# Autodesk Inventor assembly: BG003_huenin20_23
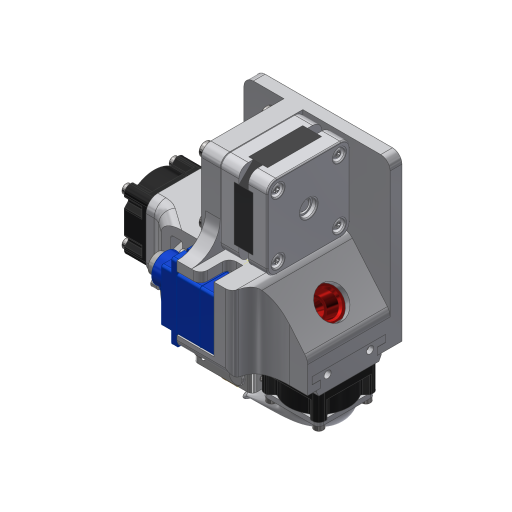
[picture p0: Inventor's stored thumbnail of the model, 512x512]
Saved by Autodesk Inventor 2023.3 (Build 273359000, 359)
## iProperties
Company: HTBLA Kaindorf
RuleStatus: InUse
Created: 2023-11-21
Part Number: BG003_huenin20_23
Project: Fiberprinter-Hotend
Material: Generisch
Description: Toolhead
Document SubType Name: Assembly
Designer: huenin20
Mass: 244.84 g
Surface Area: 631.325 cm^2
Volume: 123.223 cm^3
Density: 1.98697 g/cm^3
AfterDocNew0: iProperties-Editor_aufrufen
Author: nicob
Keywords: 2023
## Documents named in this file (17)
- H:\Dokumente\Projects\Kop\Fiberprinter_Hotend\BG003_huenin20_23_Fiberprinter-Hotend_Toolhead.iam
- H:\Dokumente\Projects\Kop\Fiberprinter_Hotend\BT010_huenin20_23_Fiberprinter-Hotend_hotendmount.ipt
- H:\Dokumente\Projects\Kop\Fiberprinter_Hotend\BT012_huenin20_23_Fiberprinter-Hotend_Faservorschubrad.ipt
- H:\Dokumente\Projects\Kop\Fiberprinter_Hotend\BT013_huenin20_23_Fiberprinter-Hotend_Faserführungsrad.ipt
- H:\Dokumente\Projects\Kop\Fiberprinter_Hotend\BT014_huenin20_23_Fiberprinter-Hotend_Faservorschubgleitlager.ipt
- H:\Dokumente\Projects\Kop\Fiberprinter_Hotend\BG001_huenin20_23_Fiberprinter-Hotend_Fiberprinter_Hotend.iam
- H:\Dokumente\Projects\Kop\Fiberprinter_Hotend\Step_downloads\Motoren\14HS08-0404S\14HS08-0404S.ipt
- H:\Dokumente\Projects\Kop\Fiberprinter_Hotend\Normteile\de-DE\ISO 2338(2)\ISO 2338 - 3 h8 x 8.ipt
- H:\Dokumente\Projects\Kop\Fiberprinter_Hotend\Step_downloads\25x25x10_fan\25x25x10_fan.ipt
- H:\Dokumente\Projects\Kop\Fiberprinter_Hotend\Step_downloads\Motoren\Servo\Servo.ipt
- H:\Dokumente\Projects\Kop\Fiberprinter_Hotend\Kurvenscheibe1.ipt
- H:\Dokumente\Projects\Kop\Fiberprinter_Hotend\Normteile\de-DE\DIN 912\DIN 912 - M3 x 0,5 x 12 x 10,75.ipt
- H:\Dokumente\Projects\Kop\Fiberprinter_Hotend\Normteile\de-DE\DIN 912\DIN 912 - M3 x 0,5 x 6 x 4,75.ipt
- H:\Dokumente\Projects\Kop\Fiberprinter_Hotend\Normteile\de-DE\ISO 4762(2)\ISO 4762 - M1,6 x 6ISO.ipt
- H:\Dokumente\Projects\Kop\Fiberprinter_Hotend\BT016_huenin20_24_Fiberprinter-Hotend_Bauteilkühllüfter_befestigung.ipt
- H:\Dokumente\Projects\Kop\Fiberprinter_Hotend\BT017_huenin20_24_Fiberprinter-Hotend_Bauteillüfterkanal.ipt
- H:\Dokumente\Projects\Kop\Fiberprinter_Hotend\Normteile\de-DE\DIN 912\DIN 912 - M2 x 0,4 x 16 x 15.ipt
## Components (30 placed, 16 different names)
1. BG001_huenin20_23_Fiberprinter-Hotend_Fiberprinter_Hotend:1 [sub-assembly] — Einfügen:61, Winkel:1, Passend:11, Winkel:2
2. DIN 912 - ersetzt durch DIN EN ISO 4762 M3 x 12:2 — Einfügen:63
3. DIN 912 - ersetzt durch DIN EN ISO 4762 M3 x 12:1 — Einfügen:62
4. DIN 912 - ersetzt durch DIN EN ISO 4762 M3 x 6:1 — Einfügen:58
5. BT010_huenin20_23_Fiberprinter-Hotend_hotendmount:1 — Einfügen:39, Einfügen:40, Einfügen:43, Einfügen:52, Einfügen:53, Einfügen:58, Einfügen:59, Einfügen:60, Einfügen:61, Winkel:1, Einfügen:62, Einfügen:63, Einfügen:64, Einfügen:65, Einfügen:66, Einfügen:67, Passend:7, Passend:8, Fluchtend:2
6. ISO 4762 M1,6 x 6:2 — Einfügen:73
7. ISO 4762 M1,6 x 6:1 — Einfügen:72
8. Servo:1 — Passend:4, Passend:5, Einfügen:59, Einfügen:60, Einfügen:72, Einfügen:73
9. Kurvenscheibe:1 — Passend:4, Passend:5
10. DIN 912 - ersetzt durch DIN EN ISO 4762 M3 x 12:6 — Einfügen:67
11. DIN 912 - ersetzt durch DIN EN ISO 4762 M3 x 12:5 — Einfügen:66
12. DIN 912 - ersetzt durch DIN EN ISO 4762 M3 x 12:4 — Einfügen:65
13. DIN 912 - ersetzt durch DIN EN ISO 4762 M3 x 12:3 — Einfügen:64
14. ISO 2338 3 h8 x 8:1 — Einfügen:44
15. BT013_huenin20_23_Fiberprinter-Hotend_Faserführungsrad:1 — Einfügen:42, Drehung:1
16. BT014_huenin20_23_Fiberprinter-Hotend_Faservorschubgleitlager:1 — Einfügen:42, Einfügen:43, Einfügen:44
17. BT012_huenin20_23_Fiberprinter-Hotend_Faservorschubrad:1 — Einfügen:41, Drehung:1
18. 14HS08-0404S:1 — Einfügen:39, Einfügen:40, Einfügen:41
19. 25x25x10_fan:1 — Einfügen:52, Einfügen:53, Einfügen:80, Einfügen:81, Einfügen:82, Einfügen:83
20. DIN 912 - ersetzt durch DIN EN ISO 4762 M2 x 16:8 — Einfügen:83
21. DIN 912 - ersetzt durch DIN EN ISO 4762 M2 x 16:6 — Einfügen:81
22. DIN 912 - ersetzt durch DIN EN ISO 4762 M2 x 16:5 — Einfügen:80
23. DIN 912 - ersetzt durch DIN EN ISO 4762 M2 x 16:7 — Einfügen:82
24. 25x25x10_fan:2 — Fluchtend:3, Passend:9, Passend:10, Einfügen:74, Einfügen:75
25. DIN 912 - ersetzt durch DIN EN ISO 4762 M2 x 16:2 — Einfügen:77
26. BT017_huenin20_24_Fiberprinter-Hotend_Bauteillüfterkanal:1 — Einfügen:74, Einfügen:75, Einfügen:76, Einfügen:77, Einfügen:78, Einfügen:79
27. DIN 912 - ersetzt durch DIN EN ISO 4762 M2 x 16:3 — Einfügen:78
28. DIN 912 - ersetzt durch DIN EN ISO 4762 M2 x 16:4 — Einfügen:79
29. DIN 912 - ersetzt durch DIN EN ISO 4762 M2 x 16:1 — Einfügen:76
30. BT016_huenin20_24_Fiberprinter-Hotend_Bauteilkühllüfter_befestigung:1 — Passend:7, Passend:8, Fluchtend:2, Fluchtend:3, Passend:9, Passend:10
## Relationships (42: Insert 30, Mate 7, Angle 2, Flush 2, RelateRotation 1)
- Einfügen:39 [Insert]: BT010_huenin20_23_Fiberprinter-Hotend_hotendmount:1 ↔ 14HS08-0404S:1
- Einfügen:40 [Insert]: BT010_huenin20_23_Fiberprinter-Hotend_hotendmount:1 ↔ 14HS08-0404S:1
- Einfügen:41 [Insert] (1 mm): BT012_huenin20_23_Fiberprinter-Hotend_Faservorschubrad:1 ↔ 14HS08-0404S:1
- Einfügen:42 [Insert]: BT013_huenin20_23_Fiberprinter-Hotend_Faserführungsrad:1 ↔ BT014_huenin20_23_Fiberprinter-Hotend_Faservorschubgleitlager:1
- Einfügen:43 [Insert]: BT010_huenin20_23_Fiberprinter-Hotend_hotendmount:1 ↔ BT014_huenin20_23_Fiberprinter-Hotend_Faservorschubgleitlager:1
- Drehung:1 [RelateRotation] (1.2 ul): BT013_huenin20_23_Fiberprinter-Hotend_Faserführungsrad:1 ↔ BT012_huenin20_23_Fiberprinter-Hotend_Faservorschubrad:1
- Einfügen:44 [Insert] (-1.5 mm): ISO 2338 3 h8 x 8:1 ↔ BT014_huenin20_23_Fiberprinter-Hotend_Faservorschubgleitlager:1
- Einfügen:52 [Insert]: BT010_huenin20_23_Fiberprinter-Hotend_hotendmount:1 ↔ 25x25x10_fan:1
- Einfügen:53 [Insert]: BT010_huenin20_23_Fiberprinter-Hotend_hotendmount:1 ↔ 25x25x10_fan:1
- Einfügen:58 [Insert]: DIN 912 - ersetzt durch DIN EN ISO 4762 M3 x 6:1 ↔ BT010_huenin20_23_Fiberprinter-Hotend_hotendmount:1
- Passend:4 [Mate]: Servo:1 ↔ Kurvenscheibe:1
- Passend:5 [Mate] (0.3 mm): Servo:1 ↔ Kurvenscheibe:1
- Einfügen:59 [Insert]: BT010_huenin20_23_Fiberprinter-Hotend_hotendmount:1 ↔ Servo:1
- Einfügen:60 [Insert]: BT010_huenin20_23_Fiberprinter-Hotend_hotendmount:1 ↔ Servo:1
- Einfügen:61 [Insert] (0.05 mm): BG001_huenin20_23_Fiberprinter-Hotend_Fiberprinter_Hotend:1 ↔ BT010_huenin20_23_Fiberprinter-Hotend_hotendmount:1
- Winkel:1 [Angle] (90 deg): BG001_huenin20_23_Fiberprinter-Hotend_Fiberprinter_Hotend:1 ↔ BT010_huenin20_23_Fiberprinter-Hotend_hotendmount:1
- Einfügen:62 [Insert]: DIN 912 - ersetzt durch DIN EN ISO 4762 M3 x 12:1 ↔ BT010_huenin20_23_Fiberprinter-Hotend_hotendmount:1
- Einfügen:63 [Insert]: DIN 912 - ersetzt durch DIN EN ISO 4762 M3 x 12:2 ↔ BT010_huenin20_23_Fiberprinter-Hotend_hotendmount:1
- Einfügen:64 [Insert]: BT010_huenin20_23_Fiberprinter-Hotend_hotendmount:1 ↔ DIN 912 - ersetzt durch DIN EN ISO 4762 M3 x 12:3
- Einfügen:65 [Insert]: BT010_huenin20_23_Fiberprinter-Hotend_hotendmount:1 ↔ DIN 912 - ersetzt durch DIN EN ISO 4762 M3 x 12:4
- Einfügen:66 [Insert]: BT010_huenin20_23_Fiberprinter-Hotend_hotendmount:1 ↔ DIN 912 - ersetzt durch DIN EN ISO 4762 M3 x 12:5
- Einfügen:67 [Insert]: BT010_huenin20_23_Fiberprinter-Hotend_hotendmount:1 ↔ DIN 912 - ersetzt durch DIN EN ISO 4762 M3 x 12:6
- Einfügen:72 [Insert]: ISO 4762 M1,6 x 6:1 ↔ Servo:1
- Einfügen:73 [Insert]: ISO 4762 M1,6 x 6:2 ↔ Servo:1
- Passend:7 [Mate]: BT010_huenin20_23_Fiberprinter-Hotend_hotendmount:1 ↔ BT016_huenin20_24_Fiberprinter-Hotend_Bauteilkühllüfter_befestigung:1
- Passend:8 [Mate]: BT010_huenin20_23_Fiberprinter-Hotend_hotendmount:1 ↔ BT016_huenin20_24_Fiberprinter-Hotend_Bauteilkühllüfter_befestigung:1
- Fluchtend:2 [Flush]: BT010_huenin20_23_Fiberprinter-Hotend_hotendmount:1 ↔ BT016_huenin20_24_Fiberprinter-Hotend_Bauteilkühllüfter_befestigung:1
- Fluchtend:3 [Flush]: 25x25x10_fan:2 ↔ BT016_huenin20_24_Fiberprinter-Hotend_Bauteilkühllüfter_befestigung:1
- Passend:9 [Mate]: 25x25x10_fan:2 ↔ BT016_huenin20_24_Fiberprinter-Hotend_Bauteilkühllüfter_befestigung:1
- Passend:10 [Mate]: 25x25x10_fan:2 ↔ BT016_huenin20_24_Fiberprinter-Hotend_Bauteilkühllüfter_befestigung:1
- Einfügen:74 [Insert]: 25x25x10_fan:2 ↔ BT017_huenin20_24_Fiberprinter-Hotend_Bauteillüfterkanal:1
- Einfügen:75 [Insert]: 25x25x10_fan:2 ↔ BT017_huenin20_24_Fiberprinter-Hotend_Bauteillüfterkanal:1
- Passend:11 [Mate]: BG001_huenin20_23_Fiberprinter-Hotend_Fiberprinter_Hotend:1
- Winkel:2 [Angle] (0 deg): BG001_huenin20_23_Fiberprinter-Hotend_Fiberprinter_Hotend:1
- Einfügen:76 [Insert]: BT017_huenin20_24_Fiberprinter-Hotend_Bauteillüfterkanal:1 ↔ DIN 912 - ersetzt durch DIN EN ISO 4762 M2 x 16:1
- Einfügen:77 [Insert]: DIN 912 - ersetzt durch DIN EN ISO 4762 M2 x 16:2 ↔ BT017_huenin20_24_Fiberprinter-Hotend_Bauteillüfterkanal:1
- Einfügen:78 [Insert]: BT017_huenin20_24_Fiberprinter-Hotend_Bauteillüfterkanal:1 ↔ DIN 912 - ersetzt durch DIN EN ISO 4762 M2 x 16:3
- Einfügen:79 [Insert]: BT017_huenin20_24_Fiberprinter-Hotend_Bauteillüfterkanal:1 ↔ DIN 912 - ersetzt durch DIN EN ISO 4762 M2 x 16:4
- Einfügen:80 [Insert]: 25x25x10_fan:1 ↔ DIN 912 - ersetzt durch DIN EN ISO 4762 M2 x 16:5
- Einfügen:81 [Insert]: 25x25x10_fan:1 ↔ DIN 912 - ersetzt durch DIN EN ISO 4762 M2 x 16:6
- Einfügen:82 [Insert]: 25x25x10_fan:1 ↔ DIN 912 - ersetzt durch DIN EN ISO 4762 M2 x 16:7
- Einfügen:83 [Insert]: 25x25x10_fan:1 ↔ DIN 912 - ersetzt durch DIN EN ISO 4762 M2 x 16:8
